# Autodesk Inventor assembly: FullAssembly
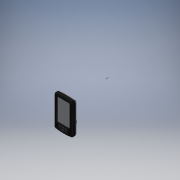
[picture p0: Inventor's stored thumbnail of the model, 180x180]
Saved by Autodesk Inventor 2018 (Build 220112000, 112)
## iProperties
Created: 2019-05-29
Part Number: FullAssembly
Document SubType Name: Assembly
Designer: Ash
Author: Ash
## Documents named in this file (8)
- C:\Autodesk\Skills 2019 Nationals\Competition\GivenFiles\Day 2 AM\Day 2 AM\FullAssembly.iam
- C:\Autodesk\Skills 2019 Nationals\Competition\AMDay2\96710A373_STAINLESS STEEL PAN HEAD TORX SCREWS.ipt
- C:\Autodesk\Skills 2019 Nationals\Competition\AMDay2\410141-1.ipt
- C:\Autodesk\Skills 2019 Nationals\Competition\AMDay2\410142.ipt
- C:\Autodesk\Skills 2019 Nationals\Competition\AMDay2\410153-1_ASM.iam
- C:\Autodesk\Skills 2019 Nationals\Competition\AMDay2\410154-1_ASSY_DISP_PMAX4.ipt
- C:\Autodesk\Skills 2019 Nationals\Competition\AMDay2\472147-1.ipt
- C:\Autodesk\Skills 2019 Nationals\Competition\AMDay2\GASKET.ipt
## Components (7 placed, 7 different names)
1. 96710A373_STAINLESS STEEL PAN HEAD TORX SCREWS:1
2. 410141-1:1 — Mate:4, Mate:5, Mate:6, Mate:7, Mate:8, Mate:9, Mate:10
3. 410142:1 — Mate:4
4. 410153-1_ASM:1 [sub-assembly] — Mate:1, Mate:2, Mate:3, Mate:9, Mate:10
5. 410154-1_ASSY_DISP_PMAX4:1 — Mate:7
6. 472147-1:1 — Mate:5, Mate:6
7. GASKET:1 — Mate:1, Mate:2, Mate:3, Mate:8
## Relationships (10: Mate 10)
- Mate:1: 410153-1_ASM:1 ↔ GASKET:1
- Mate:2: 410153-1_ASM:1 ↔ GASKET:1
- Mate:3: 410153-1_ASM:1 ↔ GASKET:1
- Mate:4: 410141-1:1 ↔ 410142:1
- Mate:5: 410141-1:1 ↔ 472147-1:1
- Mate:6: 410141-1:1 ↔ 472147-1:1
- Mate:7: 410141-1:1 ↔ 410154-1_ASSY_DISP_PMAX4:1
- Mate:8: 410141-1:1 ↔ GASKET:1
- Mate:9: 410141-1:1 ↔ 410153-1_ASM:1
- Mate:10: 410141-1:1 ↔ 410153-1_ASM:1
